# Autodesk Inventor assembly: Assembly1
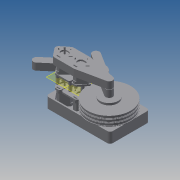
[picture p0: Inventor's stored thumbnail of the model, 180x180]
Saved by Autodesk Inventor 2013 (Build 170138000, 138)
## iProperties
Created: 2017-03-28
Part Number: Assembly1
Document SubType Name: Assembly
Designer: employee
Author: employee
## Documents named in this file (11)
- C:\Users\employee\Desktop\SCARA\Assembly1.iam
- C:\Users\employee\Desktop\SCARA\central mount.ipt
- C:\Users\employee\Desktop\SCARA\stepper.ipt
- C:\Users\employee\Desktop\SCARA\distal idler pulley.ipt
- C:\Users\employee\Desktop\SCARA\proximal drive pulley.ipt
- C:\Users\employee\Desktop\SCARA\washer.ipt
- C:\Users\employee\Desktop\SCARA\distal idler pulley special.ipt
- C:\Users\employee\Desktop\SCARA\arm.ipt
- C:\Users\employee\Desktop\SCARA\bottom plate.ipt
- C:\Users\employee\Desktop\SCARA\top plate.ipt
- C:\Users\employee\Desktop\SCARA\z idler pulley.ipt
## Components (19 placed, 10 different names)
1. central mount:1 — Insert:1, Insert:2, Insert:3, Insert:4, Angle:1, Angle:2, Angle:3, Angle:4, Mate:3
2. stepper:1 — Insert:1, Angle:1, Insert:14
3. stepper:2 — Insert:4, Angle:3, Insert:18
4. stepper:3 — Insert:3, Angle:2, Mate:1, Insert:19
5. stepper:4 — Insert:2, Angle:4, Insert:13
6. distal idler pulley:1 — Insert:8, Mate:1, Mate:2, Insert:10
7. distal idler pulley special:1 — Insert:6, Insert:7
8. proximal drive pulley:1 — Insert:9, Mate:3, Insert:12, Angle:5
9. washer:1 — Insert:6, Insert:9
10. washer:2 — Insert:7, Insert:8
11. arm:1 — Insert:12, Angle:5, Mate:4, Insert:16
12. arm:2 — Insert:11, Mate:4, Insert:15
13. washer:3 — Insert:10, Insert:11
14. bottom plate:1 — Insert:13, Insert:14
15. washer:4 — Insert:15, Insert:17
16. washer:5 — Insert:16
17. arm:3 — Insert:17, Insert:20
18. top plate:1 — Insert:18, Insert:19
19. z idler pulley:1 — Insert:20
## Relationships (28: Insert 19, Angle 5, Mate 4)
- Insert:1: central mount:1 ↔ stepper:1
- Insert:2: central mount:1 ↔ stepper:4
- Insert:3: central mount:1 ↔ stepper:3
- Insert:4: central mount:1 ↔ stepper:2
- Angle:1 (0 deg): central mount:1 ↔ stepper:1
- Angle:2 (0 deg): central mount:1 ↔ stepper:3
- Angle:3 (0 deg): central mount:1 ↔ stepper:2
- Angle:4 (0 deg): central mount:1 ↔ stepper:4
- Insert:6: distal idler pulley special:1 ↔ washer:1
- Insert:7: distal idler pulley special:1 ↔ washer:2
- Insert:8: distal idler pulley:1 ↔ washer:2
- Mate:1 (99 mm): stepper:3 ↔ distal idler pulley:1
- Insert:9: proximal drive pulley:1 ↔ washer:1
- Mate:2: distal idler pulley:1
- Mate:3 (3.4 mm): central mount:1 ↔ proximal drive pulley:1
- Insert:10: distal idler pulley:1 ↔ washer:3
- Insert:11: arm:2 ↔ washer:3
- Insert:12: proximal drive pulley:1 ↔ arm:1
- Angle:5 (0 deg): proximal drive pulley:1 ↔ arm:1
- Mate:4: arm:1 ↔ arm:2
- Insert:13: stepper:4 ↔ bottom plate:1
- Insert:14: stepper:1 ↔ bottom plate:1
- Insert:15: arm:2 ↔ washer:4
- Insert:16: arm:1 ↔ washer:5
- Insert:17: washer:4 ↔ arm:3
- Insert:18: stepper:2 ↔ top plate:1
- Insert:19: stepper:3 ↔ top plate:1
- Insert:20: arm:3 ↔ z idler pulley:1
